# Autodesk Inventor assembly: leg_bone_1_MIR
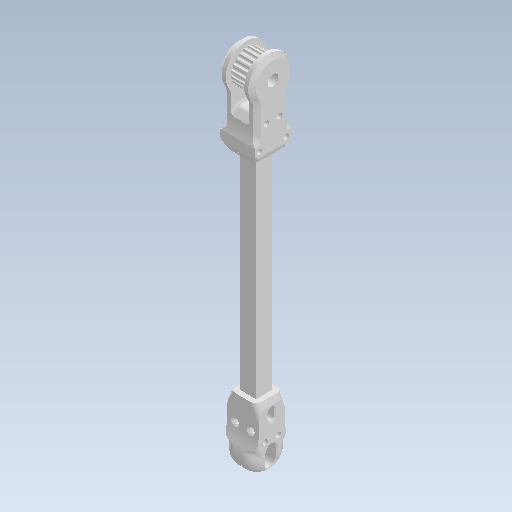
[picture p0: Inventor's stored thumbnail of the model, 512x512]
Saved by Autodesk Inventor 2020 (Build 240168000, 168)
## iProperties
Created: 2019-05-01
Part Number: leg_bone_1_MIR
Document SubType Name: Assembly
Designer: psrob
Author: psrob
## Documents named in this file (5)
- E:\projects-2\project dog gen2\hardware\leg_bone_1_MIR.iam
- E:\projects-2\project dog gen2\hardware\carbon_fiber_6_MIR.ipt
- E:\projects-2\project dog gen2\hardware\leg_down_2_MIR.ipt
- E:\projects-2\project dog gen2\hardware\leg_down_3_MIR.ipt
- E:\projects-2\project dog gen2\hardware\leg_hip_1_MIR.ipt
## Components (5 placed, 4 different names)
1. carbon_fiber_6_MIR:1 — Mate:3, Mate:2, Mate:1, Mate:5, Mate:4, Flush:1
2. leg_down_2_MIR:1 — Mate:3, Mate:2, Mate:1, Insert:2, Insert:1
3. leg_down_3_MIR:1 — Insert:2, Insert:1
4. leg_hip_1_MIR:1 — Mate:5, Mate:4, Flush:1
5. leg_hip_1_MIR:2
## Relationships (8: Mate 6, Insert 2)
- Mate:3: carbon_fiber_6_MIR:1 ↔ leg_down_2_MIR:1
- Mate:2: carbon_fiber_6_MIR:1 ↔ leg_down_2_MIR:1
- Mate:1: carbon_fiber_6_MIR:1 ↔ leg_down_2_MIR:1
- Insert:2: leg_down_2_MIR:1 ↔ leg_down_3_MIR:1
- Insert:1: leg_down_2_MIR:1 ↔ leg_down_3_MIR:1
- Mate:5: carbon_fiber_6_MIR:1 ↔ leg_hip_1_MIR:1
- Mate:4: carbon_fiber_6_MIR:1 ↔ leg_hip_1_MIR:1
- Flush:1 [Mate]: carbon_fiber_6_MIR:1 ↔ leg_hip_1_MIR:1
